# Autodesk Inventor assembly: Assembly final
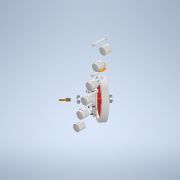
[picture p0: Inventor's stored thumbnail of the model, 180x180]
Saved by Autodesk Inventor 2020 (Build 240168000, 168)
## iProperties
Created: 2020-08-14
Part Number: Assembly final
Document SubType Name: Assembly
Designer: benny
Author: benny
## Documents named in this file (23)
- C:\Users\benny\Desktop\importantmajorprojecthev_june\engine\assembly\Assembly final.iam
- C:\Users\benny\Desktop\importantmajorprojecthev_june\engine\others\stand\stand.ipt
- C:\Users\benny\Desktop\importantmajorprojecthev_june\engine\others\bearing stand without hole.ipt
- C:\Users\benny\Documents\Inventor\Content Center Files\R2020\en-US\ISO 4762(2)\ISO 4762 - M10 x 25ISO.ipt
- C:\Users\benny\Desktop\importantmajorprojecthev_june\engine\others\bearing holder.ipt
- C:\Users\benny\Desktop\importantmajorprojecthev_june\engine\others\crank thing\crankcase.ipt
- C:\Users\benny\Desktop\importantmajorprojecthev_june\engine\assembly\Assembly2.iam
- C:\Users\benny\Documents\Inventor\Content Center Files\R2020\en-US\Parker HB 125HBL\Parker Hose Barb to Male Pipe 125HBL 125HBL-4-2.ipt
- C:\Users\benny\Desktop\importantmajorprojecthev_june\engine\others\valve housing\valve housing.ipt
- C:\Users\benny\Desktop\importantmajorprojecthev_june\engine\others\valve\valve.ipt
- C:\Users\benny\Desktop\importantmajorprojecthev_june\engine\others\connecting rod hub.ipt
- C:\Users\benny\Desktop\importantmajorprojecthev_june\engine\piston assembly\Piston Assembly.iam
- C:\Users\benny\Desktop\importantmajorprojecthev_june\engine\others\connecting rod.ipt
- C:\Users\benny\Desktop\importantmajorprojecthev_june\engine\others\crank thing\crank case cover.ipt
- C:\Users\benny\Desktop\importantmajorprojecthev_june\engine\others\crank thing\crankcase gasket.ipt
- C:\Users\benny\Documents\Inventor\Content Center Files\R2020\en-US\ISO 2338(2)\ISO 2338 - 5 h8 x 16.ipt
- C:\Users\benny\Desktop\importantmajorprojecthev_june\engine\crankshaft assembly\crankshaft assembly.iam
- C:\Users\benny\Desktop\importantmajorprojecthev_june\engine\others\flywheel not screwed.ipt
- C:\Users\benny\Documents\Inventor\Content Center Files\R2020\en-US\ISO 4762(2)\ISO 4762 - M6 x 45ISO.ipt
- C:\Users\benny\Documents\Inventor\Content Center Files\R2020\en-US\DIN 472(2)\DIN 472 - 28x1.2.ipt
- C:\Users\benny\Documents\Inventor\Content Center Files\R2020\en-US\DIN BEARING(1)\DIN 625 SKF - SKF 6001.ipt
- C:\Users\benny\Documents\Inventor\Content Center Files\R2020\en-US\ISO 7045  H\ISO 7045 - M6 x 16 - 4.8 - H - ISO.ipt
- C:\Users\benny\Documents\Inventor\Content Center Files\R2020\en-US\ISO 4028\ISO 4028 - M5 x 8 - ISO.ipt
## Components (52 placed, 22 different names)
1. stand:1 — Mate:7, Mate:8, Mate:9, Mate:10, Mate:11, Mate:12, Mate:13, Mate:14, Mate:91, Mate:93
2. bearing stand without hole:1 — Mate:18, Mate:20, Mate:72, Mate:73, Mate:93, Mate:96
3. ISO 4762 M10 x 25:1 — Mate:12, Mate:13, Mate:96
4. ISO 4762 M10 x 25:2 — Mate:11, Mate:14, Mate:91
5. ISO 4762 M10 x 25:3 — Mate:9, Mate:10, Mate:95
6. ISO 4762 M10 x 25:4 — Mate:7, Mate:8
7. bearing holder:1 — Mate:74, Mate:75, Mate:76, Mate:77, Mate:78, Mate:79, Mate:90, Mate:95
8. crankcase:1 — Mate:15, Mate:16, Mate:17, Mate:57, Flush:2, Mate:63, Mate:64, Mate:68, Mate:69, Mate:85, Mate:86, Mate:94, Mate:97
9. Parker Hose Barb to Male Pipe 125HBL 125HBL-4-2:1 — Mate:18, Mate:19, Mate:21, Mate:94
10. valve housing:1 — Mate:19, Mate:20, Mate:21, Mate:22, Mate:23, Mate:84, Mate:86
11. valve:1 — Mate:22, Mate:23
12. crank case cover:1 — Mate:62, Mate:63, Mate:64, Mate:67, Mate:87
13. crankcase gasket:1 — Mate:67, Mate:68, Mate:69, Mate:88
14. ISO 2338 5 h8 x 16:1
15. crankshaft assembly:1 [sub-assembly] — Mate:57, Flush:2, Mate:62, Mate:70, Mate:74, Mate:80, Mate:81, Mate:82, Mate:83
16. flywheel not screwed:1 — Mate:70, Mate:89, Mate:90
17. DIN 472 28x1.2:1 — Mate:75, Mate:76, Mate:77
18. DIN 625 SKF SKF 6001:1 — Mate:78, Mate:79
19. DIN 625 SKF SKF 6001:2 — Mate:82, Mate:83
20. DIN 625 SKF SKF 6001:3 — Mate:80, Mate:81
21. ISO 4028 M5 x 8:1 — Mate:89
22. connecting rod:1
23. connecting rod:2
24. connecting rod:3
25. connecting rod:4
26. connecting rod:5
27. connecting rod:6
28. connecting rod hub:1
29. Piston Assembly:1 [sub-assembly]
30. Piston Assembly:2 [sub-assembly]
31. Piston Assembly:3 [sub-assembly]
32. Piston Assembly:4 [sub-assembly]
33. Piston Assembly:5 [sub-assembly]
34. Piston Assembly:6 [sub-assembly]
35. Assembly2:6 [sub-assembly] — Mate:15, Mate:16, Mate:17
36. Assembly2:7 [sub-assembly]
37. Assembly2:8 [sub-assembly]
38. Assembly2:9 [sub-assembly]
39. Assembly2:10 [sub-assembly]
40. Assembly2:11 [sub-assembly]
41. ISO 4762 M6 x 45:1 — Mate:72, Mate:73
42. ISO 4762 M6 x 45:2 — Mate:85, Mate:97
43. ISO 4762 M6 x 45:3
44. ISO 4762 M6 x 45:4
45. ISO 4762 M6 x 45:5
46. ISO 4762 M6 x 45:6 — Mate:84
47. ISO 7045 H M6 x 16 - 4.8 - H:1 — Mate:87, Mate:88
48. ISO 7045 H M6 x 16 - 4.8 - H:2
49. ISO 7045 H M6 x 16 - 4.8 - H:3
50. ISO 7045 H M6 x 16 - 4.8 - H:4
51. ISO 7045 H M6 x 16 - 4.8 - H:5
52. ISO 7045 H M6 x 16 - 4.8 - H:6
## Component patterns: (6 elements, first: Assembly2:6), (6 elements, first: ISO 4762 M6 x 45:1), (6 elements, first: ISO 7045 H M6 x 16 - 4.8 - H:1)
## Relationships (51: Mate 50, Flush 1)
- Mate:7: stand:1 ↔ ISO 4762 M10 x 25:4
- Mate:8: stand:1 ↔ ISO 4762 M10 x 25:4
- Mate:9: stand:1 ↔ ISO 4762 M10 x 25:3
- Mate:10: stand:1 ↔ ISO 4762 M10 x 25:3
- Mate:11: stand:1 ↔ ISO 4762 M10 x 25:2
- Mate:12: stand:1 ↔ ISO 4762 M10 x 25:1
- Mate:13: stand:1 ↔ ISO 4762 M10 x 25:1
- Mate:14: stand:1 ↔ ISO 4762 M10 x 25:2
- Mate:15: crankcase:1 ↔ Assembly2:6
- Mate:16: crankcase:1 ↔ Assembly2:6
- Mate:17: crankcase:1 ↔ Assembly2:6
- Mate:18: bearing stand without hole:1 ↔ Parker Hose Barb to Male Pipe 125HBL 125HBL-4-2:1
- Mate:19: Parker Hose Barb to Male Pipe 125HBL 125HBL-4-2:1 ↔ valve housing:1
- Mate:20: bearing stand without hole:1 ↔ valve housing:1
- Mate:21: Parker Hose Barb to Male Pipe 125HBL 125HBL-4-2:1 ↔ valve housing:1
- Mate:22: valve housing:1 ↔ valve:1
- Mate:23: valve housing:1 ↔ valve:1
- Mate:57: crankcase:1 ↔ crankshaft assembly:1
- Flush:2: crankcase:1 ↔ crankshaft assembly:1
- Mate:62: crank case cover:1 ↔ crankshaft assembly:1
- Mate:63: crankcase:1 ↔ crank case cover:1
- Mate:64: crankcase:1 ↔ crank case cover:1
- Mate:67: crank case cover:1 ↔ crankcase gasket:1
- Mate:68: crankcase:1 ↔ crankcase gasket:1
- Mate:69: crankcase:1 ↔ crankcase gasket:1
- Mate:70: crankshaft assembly:1 ↔ flywheel not screwed:1
- Mate:72: bearing stand without hole:1 ↔ ISO 4762 M6 x 45:1
- Mate:73: bearing stand without hole:1 ↔ ISO 4762 M6 x 45:1
- Mate:74: bearing holder:1 ↔ crankshaft assembly:1
- Mate:75: bearing holder:1 ↔ DIN 472 28x1.2:1
- Mate:76: bearing holder:1 ↔ DIN 472 28x1.2:1
- Mate:77: bearing holder:1 ↔ DIN 472 28x1.2:1
- Mate:78: bearing holder:1 ↔ DIN 625 SKF SKF 6001:1
- Mate:79: bearing holder:1 ↔ DIN 625 SKF SKF 6001:1
- Mate:80: crankshaft assembly:1 ↔ DIN 625 SKF SKF 6001:3
- Mate:81: crankshaft assembly:1 ↔ DIN 625 SKF SKF 6001:3
- Mate:82: crankshaft assembly:1 ↔ DIN 625 SKF SKF 6001:2
- Mate:83: crankshaft assembly:1 ↔ DIN 625 SKF SKF 6001:2
- Mate:84: valve housing:1 ↔ ISO 4762 M6 x 45:6
- Mate:85: crankcase:1 ↔ ISO 4762 M6 x 45:2
- Mate:86: crankcase:1 ↔ valve housing:1
- Mate:87: crank case cover:1 ↔ ISO 7045 H M6 x 16 - 4.8 - H:1
- Mate:88: crankcase gasket:1 ↔ ISO 7045 H M6 x 16 - 4.8 - H:1
- Mate:89: flywheel not screwed:1 ↔ ISO 4028 M5 x 8:1
- Mate:90 (4 mm): bearing holder:1 ↔ flywheel not screwed:1
- Mate:91: stand:1 ↔ ISO 4762 M10 x 25:2
- Mate:93: stand:1 ↔ bearing stand without hole:1
- Mate:94: crankcase:1 ↔ Parker Hose Barb to Male Pipe 125HBL 125HBL-4-2:1
- Mate:95: ISO 4762 M10 x 25:3 ↔ bearing holder:1
- Mate:96: bearing stand without hole:1 ↔ ISO 4762 M10 x 25:1
- Mate:97: crankcase:1 ↔ ISO 4762 M6 x 45:2
